# Autodesk Inventor assembly: Shooter Assembly
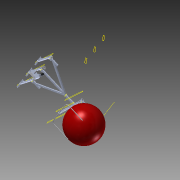
[picture p0: Inventor's stored thumbnail of the model, 180x180]
Saved by Autodesk Inventor 2014 SP1 (Build 180222100, 222)
## iProperties
Created: 2014-01-05
Part Number: Shooter Assembly
Document SubType Name: Assembly
Designer: Andrew Toennies
Mass: 1582.87 g
Surface Area: 6510.69 cm^2
Volume: 621.462 cm^3
Density: 2.54701 g/cm^3
Author: Andrew Toennies
## Documents named in this file (38)
- C:\Users\Arpan\Documents\GitHub\2014buildCAD\Shooter\Shooter Assembly.iam
- C:\Users\Arpan\Documents\GitHub\2014buildCAD\Shooter\Vex Pro 1x1 rectangular tubing 12 in length.ipt
- C:\Users\Arpan\Documents\GitHub\2014buildCAD\Shooter\Vex Pro End Bearing Mount.ipt
- C:\Users\Arpan\Documents\GitHub\2014buildCAD\Shooter\Vex Pro 1x1 rectangular tubing 27 in length.ipt
- C:\Users\Arpan\Documents\GitHub\2014buildCAD\Shooter\Vex Pro 1x1 rectangular tubing 24 in length.ipt
- C:\Users\Arpan\Documents\GitHub\2014buildCAD\Shooter\Vex Pro T gusset.ipt
- C:\Users\Arpan\Documents\GitHub\2014buildCAD\Shooter\Vex Pro Corner Gusset.ipt
- C:\Users\Arpan\Documents\GitHub\2014buildCAD\Shooter\Vex Pro 1x1 rectangular tubing 13 in length.ipt
- C:\Users\Arpan\Documents\GitHub\2014buildCAD\Shooter\Vex Pro Side Bearing Gusset.ipt
- C:\Users\Arpan\Documents\GitHub\2014buildCAD\Shooter\Bearing ID 0.500 Hex OD 1.125.ipt
- C:\Users\Arpan\Documents\GitHub\2014buildCAD\Shooter\Axle 0.500 Hex 5 in length.ipt
- C:\Users\Arpan\Documents\GitHub\2014buildCAD\Shooter\Spacer.ipt
- C:\Users\Arpan\Documents\GitHub\2014buildCAD\Shooter\Bearing ID 0.375 OD 1.125.ipt
- C:\Users\Arpan\Documents\GitHub\2014buildCAD\Shooter\Axle 0.375 3 in length.ipt
- C:\Users\Arpan\Documents\GitHub\2014buildCAD\Shooter\Vex Pro 30 tooth 9mm timing belt pulley.ipt
- C:\Users\Arpan\Documents\GitHub\2014buildCAD\Shooter\Vex Pro VersaHub 0.500 Hex.ipt
- C:\Users\Arpan\Documents\GitHub\2014buildCAD\Shooter\armbackspacer.ipt
- C:\Users\Arpan\Documents\GitHub\2014buildCAD\Shooter\Axle 0.500 Hex 3 in length.ipt
- C:\Users\Arpan\Documents\GitHub\2014buildCAD\Shooter\Worm-Drive-Gearbox-16to1.iam
- C:\Users\Arpan\Documents\GitHub\2014buildCAD\Shooter\Vex Pro 32 tooth 15 mm timing belt pulley.ipt
- C:\Users\Arpan\Documents\GitHub\2014buildCAD\Shooter\Vex Pro Traction 1 in wide 4 in dia wheel.iam
- C:\Users\Arpan\Documents\GitHub\2014buildCAD\Shooter\Aluminum Tube Bent 0.500 OD 0.436 ID.ipt
- C:\Users\Arpan\Documents\GitHub\2014buildCAD\Shooter\Bag Motor with VersaPlanetary 10 to 1 Reduction.iam
- C:\Users\Arpan\Documents\GitHub\2014buildCAD\Shooter\Vex Pro 18 tooth timing belt pulley.ipt
- C:\Users\Arpan\Documents\GitHub\2014buildCAD\Shooter\Vex Pro VersaPlanetary Face Mount.ipt
- C:\Users\Arpan\Documents\GitHub\2014buildCAD\Shooter\Foot Bracket Mount (McMaster Part #6498K710).ipt
- C:\Users\Arpan\Documents\GitHub\2014buildCAD\Shooter\Rod End (McMaster Part #6498K592).ipt
- C:\Users\Arpan\Documents\GitHub\2014buildCAD\Shooter\Spacer2.ipt
- C:\Users\Arpan\Documents\GitHub\2014buildCAD\Shooter\Bracket.ipt
- C:\Users\Arpan\Documents\GitHub\2014buildCAD\Shooter\Vex Pro 1x1 rectangular tubing 2 in length.ipt
- C:\Users\Arpan\Documents\GitHub\2014buildCAD\Shooter\Waterjetted Face Mount Bearing support VersaPlanetary.ipt
- C:\Users\Arpan\Documents\GitHub\2014buildCAD\Shooter\Axle 0.190 in 3 in length.ipt
- C:\Users\Arpan\Documents\GitHub\2014buildCAD\Shooter\Ball.ipt
- C:\Users\Arpan\Documents\GitHub\2014buildCAD\Shooter\6498K602 Pneumatic Cylinder Assembly.iam
- C:\Users\Arpan\Documents\GitHub\2014buildCAD\Shooter\bracepost.iam
- C:\Users\Arpan\Documents\GitHub\2014buildCAD\Shooter\Vex Pro 30 degree gusset.ipt
- C:\Users\Arpan\Documents\GitHub\2014buildCAD\Shooter\Vex Pro 1x1 rectangular tubing 6 in length.ipt
- C:\Users\Arpan\Documents\GitHub\2014buildCAD\Shooter\jointplate.ipt
## Components (58 placed, 37 different names)
1. Vex Pro 1x1 rectangular tubing 12 in length:1 — Flush:1, Insert:9, Insert:10, Insert:11, Insert:12, Flush:4, Mate:23, Mate:24, Mate:25, Mate:26, Mate:27, Mate:28, Mate:43, Mate:49, Mate:50, Flush:30, Flush:32, Flush:33, Mate:106, Mate:107
2. Vex Pro 1x1 rectangular tubing 27 in length:1 — Flush:1, Insert:5, Insert:6, Insert:7, Insert:8, Flush:2, Mate:2, Mate:33, Mate:34, Angle:5, Angle:6, Angle:7, Flush:34, Flush:35
3. Vex Pro 1x1 rectangular tubing 24 in length:1 — Flush:2, Mate:2, Flush:3, Mate:6, Flush:9, Mate:53, Mate:54, Flush:17, Flush:22, Flush:23, Mate:64, Mate:65, Flush:24, Mate:76, Mate:83, Mate:84, Tangent:3
4. Vex Pro T gusset:1 — Insert:5, Insert:6, Mate:6
5. Vex Pro T gusset:2 — Insert:7, Insert:8
6. Vex Pro Corner Gusset:1 — Insert:9, Insert:10
7. Vex Pro Corner Gusset:2 — Insert:11, Insert:12, Flush:31
8. Vex Pro End Bearing Mount:3 — Insert:35, Insert:47, Insert:48
9. Vex Pro End Bearing Mount:4 — Insert:36, Insert:49, Insert:50
10. Vex Pro 1x1 rectangular tubing 13 in length:1 — Flush:3, Insert:21, Insert:22, Insert:23, Insert:24, Flush:8, Flush:19, Flush:21, Mate:63, Mate:85, Mate:86, Mate:93, Flush:26, Flush:27, Flush:28, Flush:29, Angle:5
11. Vex Pro End Bearing Mount:5 — Insert:21, Insert:22, Insert:25
12. Vex Pro End Bearing Mount:6 — Insert:23, Insert:24, Insert:26
13. Bearing ID 0.500 Hex OD 1.125:1 — Insert:26, Flush:7, Mate:7, Mate:8
14. Bearing ID 0.500 Hex OD 1.125:2 — Insert:25, Flush:7, Mate:16
15. Axle 0.500 Hex 5 in length:1 — Mate:7, Mate:8, Flush:8, Mate:14, Mate:15, Mate:18, Mate:19, Mate:21, Mate:22, Flush:12, Flush:16
16. Spacer:1 — Insert:47, Insert:48, Mate:65, Flush:24
17. Spacer:2 — Insert:49, Insert:50, Flush:22, Flush:23, Mate:64
18. Bearing ID 0.375 OD 1.125:1 — Insert:35, Mate:9
19. Bearing ID 0.375 OD 1.125:2 — Insert:36, Mate:66
20. Axle 0.375 3 in length:1 — Mate:9, Flush:9, Mate:66, Mate:85
21. Vex Pro 30 tooth 9mm timing belt pulley:1 — Mate:14, Mate:15, Mate:16, Flush:18
22. Vex Pro VersaHub 0.500 Hex:1 — Mate:17, Mate:18, Mate:19, Flush:16, Insert:51, Mate:105
23. Vex Pro VersaHub 0.500 Hex:2 — Mate:17, Mate:105
24. Vex Pro VersaHub 0.500 Hex:3 — Mate:20, Mate:21, Mate:22, Flush:12, Mate:52, Insert:64
25. Vex Pro VersaHub 0.500 Hex:4 — Mate:20, Mate:52, Insert:52
26. armbackspacer:1 — Mate:26, Mate:27, Mate:28, Mate:29, Mate:30, Mate:31
27. armbackspacer:2 — Mate:23, Mate:24, Mate:25, Mate:32, Flush:13, Flush:14
28. Vex Pro Side Bearing Gusset:1 — Mate:29, Mate:30, Mate:31, Mate:35, Mate:36
29. Vex Pro Side Bearing Gusset:2 — Mate:32, Flush:13, Flush:14, Mate:37, Mate:38
30. Bearing ID 0.500 Hex OD 1.125:3 — Mate:35, Mate:36
31. Axle 0.500 Hex 3 in length:1 — Mate:33, Mate:34, Mate:39, Mate:40, Flush:15, Mate:47, Mate:48
32. Bearing ID 0.500 Hex OD 1.125:4 — Mate:37, Mate:38, Mate:39, Mate:40, Flush:15
33. Worm-Drive-Gearbox-16to1:1 [sub-assembly] — Mate:43, Mate:49, Mate:50
34. Vex Pro 32 tooth 15 mm timing belt pulley:1 — Mate:47, Mate:48
35. Vex Pro Traction 1 in wide 4 in dia wheel:1 [sub-assembly] — Insert:51, Mate:98
36. Vex Pro Traction 1 in wide 4 in dia wheel:2 [sub-assembly] — Insert:52, Insert:64
37. Aluminum Tube Bent 0.500 OD 0.436 ID:1 — Mate:53, Mate:54, Flush:17, Tangent:1, Tangent:2
38. Bag Motor with VersaPlanetary 10 to 1 Reduction:1 [sub-assembly] — Mate:55, Mate:56, Flush:19, Insert:53, Insert:54, Angle:4
39. Vex Pro 18 tooth timing belt pulley:1 — Mate:55, Mate:56, Flush:18
40. Vex Pro VersaPlanetary Face Mount:1 — Insert:53, Insert:54, Flush:21, Mate:63, Mate:77, Mate:78, Mate:79
41. Foot Bracket Mount (McMaster Part #6498K710):1 — Mate:71, Mate:72, Mate:73, Mate:99, Mate:100
42. Rod End (McMaster Part #6498K592):1 — Mate:102, Mate:103
43. Spacer2:1 — Mate:71, Mate:72, Mate:73, Mate:76, Mate:83, Mate:84
44. Bracket:1 — Mate:93, Mate:96, Flush:25, Flush:28, Flush:29
45. Bracket:2 — Mate:86, Mate:97, Flush:26, Flush:27
46. Vex Pro 1x1 rectangular tubing 2 in length:1 — Mate:77, Mate:78, Mate:79, Mate:80, Mate:81, Mate:82
47. Waterjetted Face Mount Bearing support VersaPlanetary:1 — Mate:80, Mate:81, Mate:82, Insert:63
48. Bearing ID 0.500 Hex OD 1.125:5 — Insert:63, Angle:4
49. Axle 0.190 in 3 in length:1 — Mate:96, Mate:97, Flush:25, Mate:103
50. Ball:1 — Tangent:1, Tangent:2, Tangent:3
51. 6498K602 Pneumatic Cylinder Assembly:1 [sub-assembly] — Mate:99, Mate:100, Mate:102
52. bracepost:1 [sub-assembly] — Flush:32, Flush:33, Angle:6, Mate:107, Mate:108, Mate:110, Mate:111, Mate:119
53. bracepost:2 [sub-assembly] — Flush:30, Flush:31, Angle:7, Mate:106, Mate:113, Mate:114, Mate:115
54. Vex Pro 30 degree gusset:1 — Mate:108, Mate:110, Mate:111, Mate:120
55. Vex Pro 30 degree gusset:2 — Mate:113, Mate:114, Mate:115, Mate:116, Mate:117, Mate:118
56. Vex Pro 1x1 rectangular tubing 6 in length:1 — Mate:116, Mate:117, Mate:118
57. Vex Pro 1x1 rectangular tubing 6 in length:2 — Flush:34, Mate:119, Mate:120
58. jointplate:1 — Flush:35
## Relationships (146: Mate 82, Flush 31, Insert 26, Angle 4, Tangent 3)
- Flush:1: Vex Pro 1x1 rectangular tubing 12 in length:1 ↔ Vex Pro 1x1 rectangular tubing 27 in length:1
- Insert:5: Vex Pro 1x1 rectangular tubing 27 in length:1 ↔ Vex Pro T gusset:1
- Insert:6: Vex Pro 1x1 rectangular tubing 27 in length:1 ↔ Vex Pro T gusset:1
- Insert:7: Vex Pro 1x1 rectangular tubing 27 in length:1 ↔ Vex Pro T gusset:2
- Insert:8: Vex Pro 1x1 rectangular tubing 27 in length:1 ↔ Vex Pro T gusset:2
- Flush:2: Vex Pro 1x1 rectangular tubing 27 in length:1 ↔ Vex Pro 1x1 rectangular tubing 24 in length:1
- Mate:2: Vex Pro 1x1 rectangular tubing 27 in length:1 ↔ Vex Pro 1x1 rectangular tubing 24 in length:1
- Insert:9: Vex Pro 1x1 rectangular tubing 12 in length:1 ↔ Vex Pro Corner Gusset:1
- Insert:10: Vex Pro 1x1 rectangular tubing 12 in length:1 ↔ Vex Pro Corner Gusset:1
- Insert:11: Vex Pro 1x1 rectangular tubing 12 in length:1 ↔ Vex Pro Corner Gusset:2
- Insert:12: Vex Pro 1x1 rectangular tubing 12 in length:1 ↔ Vex Pro Corner Gusset:2
- Flush:3: Vex Pro 1x1 rectangular tubing 24 in length:1 ↔ Vex Pro 1x1 rectangular tubing 13 in length:1
- Flush:4: Vex Pro 1x1 rectangular tubing 12 in length:1
- Mate:6: Vex Pro 1x1 rectangular tubing 24 in length:1 ↔ Vex Pro T gusset:1
- Flush:5 (-711.2 mm)
- Insert:21: Vex Pro 1x1 rectangular tubing 13 in length:1 ↔ Vex Pro End Bearing Mount:5
- Insert:22: Vex Pro 1x1 rectangular tubing 13 in length:1 ↔ Vex Pro End Bearing Mount:5
- Insert:23: Vex Pro 1x1 rectangular tubing 13 in length:1 ↔ Vex Pro End Bearing Mount:6
- Insert:24: Vex Pro 1x1 rectangular tubing 13 in length:1 ↔ Vex Pro End Bearing Mount:6
- Insert:25: Vex Pro End Bearing Mount:5 ↔ Bearing ID 0.500 Hex OD 1.125:2
- Insert:26: Vex Pro End Bearing Mount:6 ↔ Bearing ID 0.500 Hex OD 1.125:1
- Flush:7: Bearing ID 0.500 Hex OD 1.125:1 ↔ Bearing ID 0.500 Hex OD 1.125:2
- Mate:7: Bearing ID 0.500 Hex OD 1.125:1 ↔ Axle 0.500 Hex 5 in length:1
- Mate:8: Bearing ID 0.500 Hex OD 1.125:1 ↔ Axle 0.500 Hex 5 in length:1
- Flush:8 (-63.5 mm): Vex Pro 1x1 rectangular tubing 13 in length:1 ↔ Axle 0.500 Hex 5 in length:1
- Insert:35: Vex Pro End Bearing Mount:3 ↔ Bearing ID 0.375 OD 1.125:1
- Insert:36: Vex Pro End Bearing Mount:4 ↔ Bearing ID 0.375 OD 1.125:2
- Mate:9: Bearing ID 0.375 OD 1.125:1 ↔ Axle 0.375 3 in length:1
- Flush:9 (-25.4 mm): Vex Pro 1x1 rectangular tubing 24 in length:1 ↔ Axle 0.375 3 in length:1
- Mate:14: Axle 0.500 Hex 5 in length:1 ↔ Vex Pro 30 tooth 9mm timing belt pulley:1
- Mate:15: Axle 0.500 Hex 5 in length:1 ↔ Vex Pro 30 tooth 9mm timing belt pulley:1
- Mate:16: Bearing ID 0.500 Hex OD 1.125:2 ↔ Vex Pro 30 tooth 9mm timing belt pulley:1
- Mate:17: Vex Pro VersaHub 0.500 Hex:1 ↔ Vex Pro VersaHub 0.500 Hex:2
- Mate:18: Axle 0.500 Hex 5 in length:1 ↔ Vex Pro VersaHub 0.500 Hex:1
- Mate:19: Axle 0.500 Hex 5 in length:1 ↔ Vex Pro VersaHub 0.500 Hex:1
- Mate:20: Vex Pro VersaHub 0.500 Hex:3 ↔ Vex Pro VersaHub 0.500 Hex:4
- Mate:21: Axle 0.500 Hex 5 in length:1 ↔ Vex Pro VersaHub 0.500 Hex:3
- Mate:22: Axle 0.500 Hex 5 in length:1 ↔ Vex Pro VersaHub 0.500 Hex:3
- Flush:12 (9.525 mm): Axle 0.500 Hex 5 in length:1 ↔ Vex Pro VersaHub 0.500 Hex:3
- Mate:23: Vex Pro 1x1 rectangular tubing 12 in length:1 ↔ armbackspacer:2
- Mate:24: Vex Pro 1x1 rectangular tubing 12 in length:1 ↔ armbackspacer:2
- Mate:25: Vex Pro 1x1 rectangular tubing 12 in length:1 ↔ armbackspacer:2
- Mate:26: Vex Pro 1x1 rectangular tubing 12 in length:1 ↔ armbackspacer:1
- Mate:27: Vex Pro 1x1 rectangular tubing 12 in length:1 ↔ armbackspacer:1
- Mate:28: Vex Pro 1x1 rectangular tubing 12 in length:1 ↔ armbackspacer:1
- Mate:29: armbackspacer:1 ↔ Vex Pro Side Bearing Gusset:1
- Mate:30: armbackspacer:1 ↔ Vex Pro Side Bearing Gusset:1
- Mate:31: armbackspacer:1 ↔ Vex Pro Side Bearing Gusset:1
- Mate:32: armbackspacer:2 ↔ Vex Pro Side Bearing Gusset:2
- Flush:13: armbackspacer:2 ↔ Vex Pro Side Bearing Gusset:2
- Flush:14: armbackspacer:2 ↔ Vex Pro Side Bearing Gusset:2
- Mate:33: Vex Pro 1x1 rectangular tubing 27 in length:1 ↔ Axle 0.500 Hex 3 in length:1
- Mate:34: Vex Pro 1x1 rectangular tubing 27 in length:1 ↔ Axle 0.500 Hex 3 in length:1
- Mate:35: Vex Pro Side Bearing Gusset:1 ↔ Bearing ID 0.500 Hex OD 1.125:3
- Mate:36: Vex Pro Side Bearing Gusset:1 ↔ Bearing ID 0.500 Hex OD 1.125:3
- Mate:37: Vex Pro Side Bearing Gusset:2 ↔ Bearing ID 0.500 Hex OD 1.125:4
- Mate:38: Vex Pro Side Bearing Gusset:2 ↔ Bearing ID 0.500 Hex OD 1.125:4
- Mate:39: Axle 0.500 Hex 3 in length:1 ↔ Bearing ID 0.500 Hex OD 1.125:4
- Mate:40: Axle 0.500 Hex 3 in length:1 ↔ Bearing ID 0.500 Hex OD 1.125:4
- Flush:15 (-9.525 mm): Axle 0.500 Hex 3 in length:1 ↔ Bearing ID 0.500 Hex OD 1.125:4
- Flush:16 (12.7 mm): Axle 0.500 Hex 5 in length:1 ↔ Vex Pro VersaHub 0.500 Hex:1
- Mate:43: Vex Pro 1x1 rectangular tubing 12 in length:1 ↔ Worm-Drive-Gearbox-16to1:1
- Mate:47: Axle 0.500 Hex 3 in length:1 ↔ Vex Pro 32 tooth 15 mm timing belt pulley:1
- Mate:48: Axle 0.500 Hex 3 in length:1 ↔ Vex Pro 32 tooth 15 mm timing belt pulley:1
- Mate:49: Vex Pro 1x1 rectangular tubing 12 in length:1 ↔ Worm-Drive-Gearbox-16to1:1
- Mate:50: Vex Pro 1x1 rectangular tubing 12 in length:1 ↔ Worm-Drive-Gearbox-16to1:1
- Insert:47: Vex Pro End Bearing Mount:3 ↔ Spacer:1
- Insert:48: Vex Pro End Bearing Mount:3 ↔ Spacer:1
- Insert:49: Vex Pro End Bearing Mount:4 ↔ Spacer:2
- Insert:50: Vex Pro End Bearing Mount:4 ↔ Spacer:2
- Mate:52: Vex Pro VersaHub 0.500 Hex:3 ↔ Vex Pro VersaHub 0.500 Hex:4
- Insert:51: Vex Pro VersaHub 0.500 Hex:1 ↔ Vex Pro Traction 1 in wide 4 in dia wheel:1
- Insert:52: Vex Pro VersaHub 0.500 Hex:4 ↔ Vex Pro Traction 1 in wide 4 in dia wheel:2
- Mate:53: Vex Pro 1x1 rectangular tubing 24 in length:1 ↔ Aluminum Tube Bent 0.500 OD 0.436 ID:1
- Mate:54 (196.85 mm): Vex Pro 1x1 rectangular tubing 24 in length:1 ↔ Aluminum Tube Bent 0.500 OD 0.436 ID:1
- Flush:17 (323.85 mm): Vex Pro 1x1 rectangular tubing 24 in length:1 ↔ Aluminum Tube Bent 0.500 OD 0.436 ID:1
- Mate:55: Bag Motor with VersaPlanetary 10 to 1 Reduction:1 ↔ Vex Pro 18 tooth timing belt pulley:1
- Mate:56: Bag Motor with VersaPlanetary 10 to 1 Reduction:1 ↔ Vex Pro 18 tooth timing belt pulley:1
- Flush:18: Vex Pro 30 tooth 9mm timing belt pulley:1 ↔ Vex Pro 18 tooth timing belt pulley:1
- Flush:19: Vex Pro 1x1 rectangular tubing 13 in length:1 ↔ Bag Motor with VersaPlanetary 10 to 1 Reduction:1
- Insert:53: Bag Motor with VersaPlanetary 10 to 1 Reduction:1 ↔ Vex Pro VersaPlanetary Face Mount:1
- Insert:54: Bag Motor with VersaPlanetary 10 to 1 Reduction:1 ↔ Vex Pro VersaPlanetary Face Mount:1
- Flush:21: Vex Pro 1x1 rectangular tubing 13 in length:1 ↔ Vex Pro VersaPlanetary Face Mount:1
- Mate:63: Vex Pro 1x1 rectangular tubing 13 in length:1 ↔ Vex Pro VersaPlanetary Face Mount:1
- Flush:22: Vex Pro 1x1 rectangular tubing 24 in length:1 ↔ Spacer:2
- Flush:23: Vex Pro 1x1 rectangular tubing 24 in length:1 ↔ Spacer:2
- Mate:64: Vex Pro 1x1 rectangular tubing 24 in length:1 ↔ Spacer:2
- Mate:65: Vex Pro 1x1 rectangular tubing 24 in length:1 ↔ Spacer:1
- Flush:24: Vex Pro 1x1 rectangular tubing 24 in length:1 ↔ Spacer:1
- Mate:66: Bearing ID 0.375 OD 1.125:2 ↔ Axle 0.375 3 in length:1
- Mate:71: Foot Bracket Mount (McMaster Part #6498K710):1 ↔ Spacer2:1
- Mate:72: Foot Bracket Mount (McMaster Part #6498K710):1 ↔ Spacer2:1
- Mate:73: Foot Bracket Mount (McMaster Part #6498K710):1 ↔ Spacer2:1
- Mate:76: Vex Pro 1x1 rectangular tubing 24 in length:1 ↔ Spacer2:1
- Mate:77: Vex Pro VersaPlanetary Face Mount:1 ↔ Vex Pro 1x1 rectangular tubing 2 in length:1
- Mate:78: Vex Pro VersaPlanetary Face Mount:1 ↔ Vex Pro 1x1 rectangular tubing 2 in length:1
- Mate:79: Vex Pro VersaPlanetary Face Mount:1 ↔ Vex Pro 1x1 rectangular tubing 2 in length:1
- Mate:80: Vex Pro 1x1 rectangular tubing 2 in length:1 ↔ Waterjetted Face Mount Bearing support VersaPlanetary:1
- Mate:81: Vex Pro 1x1 rectangular tubing 2 in length:1 ↔ Waterjetted Face Mount Bearing support VersaPlanetary:1
- Mate:82: Vex Pro 1x1 rectangular tubing 2 in length:1 ↔ Waterjetted Face Mount Bearing support VersaPlanetary:1
- Insert:63: Waterjetted Face Mount Bearing support VersaPlanetary:1 ↔ Bearing ID 0.500 Hex OD 1.125:5
- Angle:4 (0 deg): Bag Motor with VersaPlanetary 10 to 1 Reduction:1 ↔ Bearing ID 0.500 Hex OD 1.125:5
- Mate:83: Vex Pro 1x1 rectangular tubing 24 in length:1 ↔ Spacer2:1
- Mate:84: Vex Pro 1x1 rectangular tubing 24 in length:1 ↔ Spacer2:1
- Insert:64: Vex Pro VersaHub 0.500 Hex:3 ↔ Vex Pro Traction 1 in wide 4 in dia wheel:2
- Mate:85: Vex Pro 1x1 rectangular tubing 13 in length:1 ↔ Axle 0.375 3 in length:1
- Mate:86: Vex Pro 1x1 rectangular tubing 13 in length:1 ↔ Bracket:2
- Mate:93: Vex Pro 1x1 rectangular tubing 13 in length:1 ↔ Bracket:1
- Mate:96: Bracket:1 ↔ Axle 0.190 in 3 in length:1
- Mate:97: Bracket:2 ↔ Axle 0.190 in 3 in length:1
- Flush:25 (-11.1125 mm): Bracket:1 ↔ Axle 0.190 in 3 in length:1
- Tangent:1: Aluminum Tube Bent 0.500 OD 0.436 ID:1 ↔ Ball:1
- Tangent:2: Aluminum Tube Bent 0.500 OD 0.436 ID:1 ↔ Ball:1
- Tangent:3 (12.7 mm): Vex Pro 1x1 rectangular tubing 24 in length:1 ↔ Ball:1
- Mate:98: Vex Pro Traction 1 in wide 4 in dia wheel:1
- Flush:26: Vex Pro 1x1 rectangular tubing 13 in length:1 ↔ Bracket:2
- Flush:27 (109.22 mm): Vex Pro 1x1 rectangular tubing 13 in length:1 ↔ Bracket:2
- Flush:28 (109.22 mm): Vex Pro 1x1 rectangular tubing 13 in length:1 ↔ Bracket:1
- Flush:29: Vex Pro 1x1 rectangular tubing 13 in length:1 ↔ Bracket:1
- Mate:99: Foot Bracket Mount (McMaster Part #6498K710):1 ↔ 6498K602 Pneumatic Cylinder Assembly:1
- Mate:100: Foot Bracket Mount (McMaster Part #6498K710):1 ↔ 6498K602 Pneumatic Cylinder Assembly:1
- Mate:102: Rod End (McMaster Part #6498K592):1 ↔ 6498K602 Pneumatic Cylinder Assembly:1
- Mate:103: Rod End (McMaster Part #6498K592):1 ↔ Axle 0.190 in 3 in length:1
- Mate:105: Vex Pro VersaHub 0.500 Hex:1 ↔ Vex Pro VersaHub 0.500 Hex:2
- Angle:5 (1.4 deg): Vex Pro 1x1 rectangular tubing 27 in length:1 ↔ Vex Pro 1x1 rectangular tubing 13 in length:1
- Flush:30: Vex Pro 1x1 rectangular tubing 12 in length:1 ↔ bracepost:2
- Flush:31: Vex Pro Corner Gusset:2 ↔ bracepost:2
- Flush:32: Vex Pro 1x1 rectangular tubing 12 in length:1 ↔ bracepost:1
- Flush:33: Vex Pro 1x1 rectangular tubing 12 in length:1 ↔ bracepost:1
- Angle:6 (0 deg): Vex Pro 1x1 rectangular tubing 27 in length:1 ↔ bracepost:1
- Angle:7 (0 deg): Vex Pro 1x1 rectangular tubing 27 in length:1 ↔ bracepost:2
- Mate:106 (228.6 mm): Vex Pro 1x1 rectangular tubing 12 in length:1 ↔ bracepost:2
- Mate:107 (228.6 mm): Vex Pro 1x1 rectangular tubing 12 in length:1 ↔ bracepost:1
- Mate:108: bracepost:1 ↔ Vex Pro 30 degree gusset:1
- Mate:110: bracepost:1 ↔ Vex Pro 30 degree gusset:1
- Mate:111: bracepost:1 ↔ Vex Pro 30 degree gusset:1
- Mate:113: bracepost:2 ↔ Vex Pro 30 degree gusset:2
- Mate:114: bracepost:2 ↔ Vex Pro 30 degree gusset:2
- Mate:115: bracepost:2 ↔ Vex Pro 30 degree gusset:2
- Mate:116: Vex Pro 30 degree gusset:2 ↔ Vex Pro 1x1 rectangular tubing 6 in length:1
- Mate:117: Vex Pro 30 degree gusset:2 ↔ Vex Pro 1x1 rectangular tubing 6 in length:1
- Mate:118: Vex Pro 30 degree gusset:2 ↔ Vex Pro 1x1 rectangular tubing 6 in length:1
- Flush:34: Vex Pro 1x1 rectangular tubing 27 in length:1 ↔ Vex Pro 1x1 rectangular tubing 6 in length:2
- Mate:119: bracepost:1 ↔ Vex Pro 1x1 rectangular tubing 6 in length:2
- Mate:120: Vex Pro 30 degree gusset:1 ↔ Vex Pro 1x1 rectangular tubing 6 in length:2
- Flush:35: Vex Pro 1x1 rectangular tubing 27 in length:1 ↔ jointplate:1
